# Autodesk Inventor assembly: Ensamblaje
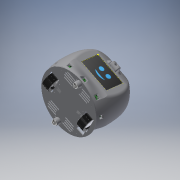
[picture p0: Inventor's stored thumbnail of the model, 180x180]
Saved by Autodesk Inventor 2018 (Build 220112000, 112)
## iProperties
Created: 2018-07-25
Part Number: Ensamblaje
Material: Genérico
Document SubType Name: Assembly
Designer: ivanb
Author: ivanb
## Documents named in this file (19)
- \\VBOXSVR\tranmision_de_archivos\learnbot-git-annex\learnbot_desings\Learnbot2.2\IPT\Ensamblaje.iam
- \\VBOXSVR\tranmision_de_archivos\learnbot-git-annex\learnbot_desings\Learnbot2.2\IPT\Base.ipt
- \\VBOXSVR\tranmision_de_archivos\learnbot-git-annex\learnbot_desings\Learnbot2.2\IPT\BackCase.ipt
- \\VBOXSVR\tranmision_de_archivos\learnbot-git-annex\learnbot_desings\Learnbot2.2\IPT\Front Case.ipt
- \\VBOXSVR\tranmision_de_archivos\learnbot-git-annex\learnbot_desings\Learnbot2.2\IPT\Pitft 3.5.ipt
- \\VBOXSVR\tranmision_de_archivos\learnbot-git-annex\learnbot_desings\Learnbot2.2\IPT\Laser.ipt
- \\VBOXSVR\tranmision_de_archivos\learnbot-git-annex\learnbot_desings\Learnbot2.2\IPT\servo motor.ipt
- \\VBOXSVR\tranmision_de_archivos\learnbot-git-annex\learnbot_desings\Learnbot2.2\IPT\servo pulley.ipt
- \\VBOXSVR\tranmision_de_archivos\learnbot-git-annex\learnbot_desings\Learnbot2.2\IPT\Soport Raspberry.ipt
- \\VBOXSVR\tranmision_de_archivos\learnbot-git-annex\learnbot_desings\Learnbot2.2\IPT\raspberrypi.ipt
- \\VBOXSVR\tranmision_de_archivos\learnbot-git-annex\learnbot_desings\Learnbot2.2\IPT\Wheel.ipt
- \\VBOXSVR\tranmision_de_archivos\learnbot-git-annex\learnbot_desings\Learnbot2.2\IPT\d24v50f5-step-down-voltage-regulator.ipt
- \\VBOXSVR\tranmision_de_archivos\learnbot-git-annex\learnbot_desings\Learnbot2.2\IPT\drv8835-dual-motor-driver-carrier.ipt
- \\VBOXSVR\tranmision_de_archivos\learnbot-git-annex\learnbot_desings\Learnbot2.2\IPT\CameraCase.ipt
- \\VBOXSVR\tranmision_de_archivos\learnbot-git-annex\learnbot_desings\Learnbot2.2\IPT\spacer 3mm.ipt
- \\VBOXSVR\tranmision_de_archivos\learnbot-git-annex\learnbot_desings\Learnbot2.2\IPT\Board 16 pwm.ipt
- \\VBOXSVR\tranmision_de_archivos\learnbot-git-annex\learnbot_desings\Learnbot2.2\IPT\Shield.ipt
- \\VBOXSVR\tranmision_de_archivos\learnbot-git-annex\learnbot_desings\Learnbot2.2\IPT\ball.ipt
- \\VBOXSVR\tranmision_de_archivos\EBO_definitivo\IPT\displaysuport.ipt
## Components (29 placed, 18 different names)
1. Base:1 — Insertar:1, Insertar:2, Insertar:3, Insertar:4, Insertar:28, Insertar:29, Nivelación:1, Nivelación:2, Insertar:38, Insertar:39
2. BackCase:1 — Insertar:1, Insertar:2
3. Front Case:1 — Insertar:3, Insertar:4, Coincidencia:1, Coincidencia:2, Coincidencia:3, Insertar:5, Insertar:6, Insertar:8, Insertar:9, Insertar:10, Insertar:11, Insertar:13, Insertar:14, Insertar:15, Insertar:16, De rotación:1, Insertar:32, Insertar:33, Nivelación:3, Insertar:40, Insertar:41
4. Pitft 3.5:1 — Coincidencia:1, Coincidencia:2, Coincidencia:3
5. Laser:1 — Insertar:40, Insertar:41
6. Laser:2 — Insertar:8, Insertar:13
7. Laser:3 — Insertar:5, Insertar:11
8. Laser:4 — Insertar:6, Insertar:10
9. Laser:5 — Insertar:9, Insertar:14
10. servo motor:1 — Insertar:15, Insertar:16, Insertar:17
11. servo pulley:1 — Insertar:17
12. raspberrypi:1 — Insertar:22, Insertar:23, Insertar:26, Insertar:27, Coincidencia:7, Coincidencia:8, Coincidencia:9
13. Wheel:1 — Rígido:1
14. Wheel:2 — Rígido:2
15. drv8835-dual-motor-driver-carrier:1 — Coincidencia:10, Coincidencia:11, Nivelación:6
16. CameraCase:1 — De rotación:1
17. spacer 3mm:2 — Insertar:37
18. spacer 3mm:3 — Insertar:36
19. spacer 3mm:4 — Insertar:23, Insertar:31
20. spacer 3mm:5 — Insertar:26
21. spacer 3mm:6 — Insertar:27, Insertar:30
22. spacer 3mm:7 — Insertar:22
23. Soport Raspberry:1 — Rígido:1, Rígido:2, Insertar:28, Insertar:29, Insertar:30, Insertar:31, Insertar:36, Insertar:37
24. Board 16 pwm:1 — Insertar:32, Insertar:33
25. Shield:1 — Coincidencia:7, Coincidencia:8, Coincidencia:9, Coincidencia:10, Coincidencia:11, Coincidencia:12, Nivelación:4, Nivelación:5, Nivelación:6
26. d24v50f5-step-down-voltage-regulator:1 — Coincidencia:12, Nivelación:4, Nivelación:5
27. ball:1 — Nivelación:1, Nivelación:2
28. ball:2 — Insertar:38, Insertar:39
29. displaysuport:1 — Nivelación:3
## Relationships (49: Insert 31, Mate 9, Flush 6, WeldJoint 2, RevoluteJoint 1)
- Insertar:1: Base:1 ↔ BackCase:1
- Insertar:2: Base:1 ↔ BackCase:1
- Insertar:3: Base:1 ↔ Front Case:1
- Insertar:4: Base:1 ↔ Front Case:1
- Coincidencia:1 [Mate]: Front Case:1 ↔ Pitft 3.5:1
- Coincidencia:2 [Mate]: Front Case:1 ↔ Pitft 3.5:1
- Coincidencia:3 [Mate]: Front Case:1 ↔ Pitft 3.5:1
- Insertar:5: Front Case:1 ↔ Laser:3
- Insertar:6: Front Case:1 ↔ Laser:4
- Insertar:8: Front Case:1 ↔ Laser:2
- Insertar:9: Front Case:1 ↔ Laser:5
- Insertar:10: Front Case:1 ↔ Laser:4
- Insertar:11: Front Case:1 ↔ Laser:3
- Insertar:13: Front Case:1 ↔ Laser:2
- Insertar:14: Front Case:1 ↔ Laser:5
- Insertar:15: Front Case:1 ↔ servo motor:1
- Insertar:16: Front Case:1 ↔ servo motor:1
- Insertar:17 (0.7 mm): servo motor:1 ↔ servo pulley:1
- De rotación:1 [RevoluteJoint] (-1 mm): Front Case:1 ↔ CameraCase:1
- Insertar:22: raspberrypi:1 ↔ spacer 3mm:7
- Insertar:23: raspberrypi:1 ↔ spacer 3mm:4
- Insertar:26: raspberrypi:1 ↔ spacer 3mm:5
- Insertar:27: raspberrypi:1 ↔ spacer 3mm:6
- Rígido:1 [WeldJoint]: Wheel:1 ↔ Soport Raspberry:1
- Rígido:2 [WeldJoint]: Wheel:2 ↔ Soport Raspberry:1
- Insertar:28: Base:1 ↔ Soport Raspberry:1
- Insertar:29: Base:1 ↔ Soport Raspberry:1
- Insertar:30: spacer 3mm:6 ↔ Soport Raspberry:1
- Insertar:31: spacer 3mm:4 ↔ Soport Raspberry:1
- Insertar:32: Front Case:1 ↔ Board 16 pwm:1
- Insertar:33: Front Case:1 ↔ Board 16 pwm:1
- Coincidencia:7 [Mate]: raspberrypi:1 ↔ Shield:1
- Coincidencia:8 [Mate]: raspberrypi:1 ↔ Shield:1
- Coincidencia:9 [Mate]: raspberrypi:1 ↔ Shield:1
- Coincidencia:10 [Mate] (2 mm): drv8835-dual-motor-driver-carrier:1 ↔ Shield:1
- Coincidencia:11 [Mate] (-32 mm): drv8835-dual-motor-driver-carrier:1 ↔ Shield:1
- Insertar:36: spacer 3mm:3 ↔ Soport Raspberry:1
- Insertar:37: spacer 3mm:2 ↔ Soport Raspberry:1
- Nivelación:1 [Flush]: Base:1 ↔ ball:1
- Nivelación:2 [Flush]: Base:1 ↔ ball:1
- Insertar:38: Base:1 ↔ ball:2
- Insertar:39: Base:1 ↔ ball:2
- Nivelación:3 [Flush]: Front Case:1 ↔ displaysuport:1
- Insertar:40: Front Case:1 ↔ Laser:1
- Insertar:41: Front Case:1 ↔ Laser:1
- Coincidencia:12 [Mate] (3 mm): Shield:1 ↔ d24v50f5-step-down-voltage-regulator:1
- Nivelación:4 [Flush] (2.5 mm): Shield:1 ↔ d24v50f5-step-down-voltage-regulator:1
- Nivelación:5 [Flush] (33.5 mm): Shield:1 ↔ d24v50f5-step-down-voltage-regulator:1
- Nivelación:6 [Flush] (2.5 mm): drv8835-dual-motor-driver-carrier:1 ↔ Shield:1
